# Autodesk Inventor assembly: AlBlankAssy
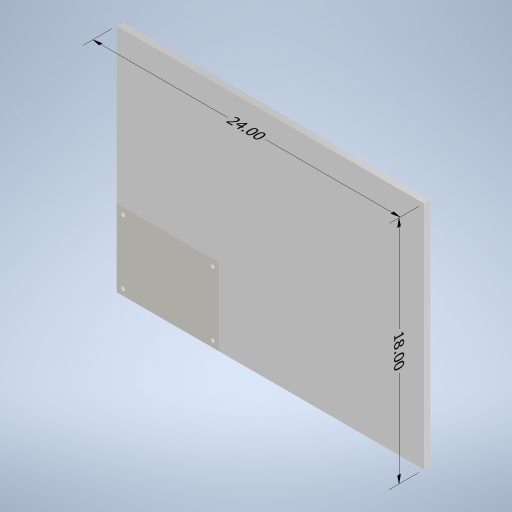
[picture p0: Inventor's stored thumbnail of the model, 512x512]
Saved by Autodesk Inventor 2023 (Build 270158000, 158)
## iProperties
Created: 2022-12-05
Part Number: AlBlankAssy
Document SubType Name: Assembly
Designer: 223076749
Author: 223076749
## Documents named in this file (3)
- C:\Users\223076749\Documents\AlBlankAssy.iam
- C:\Users\223076749\Documents\AlBlank.ipt
- C:\Users\223076749\Documents\Discrete Demo 2023\Base Plate.ipt
## Components (2 placed, 2 different names)
1. AlBlank:1 — Flush:1, Flush:2, Flush:3
2. Base Plate:1 — Flush:1, Flush:2, Flush:3
## Relationships (3: Flush 3)
- Flush:1: AlBlank:1 ↔ Base Plate:1
- Flush:2: AlBlank:1 ↔ Base Plate:1
- Flush:3: AlBlank:1 ↔ Base Plate:1
